# Autodesk Inventor assembly: UBG-Antrieb
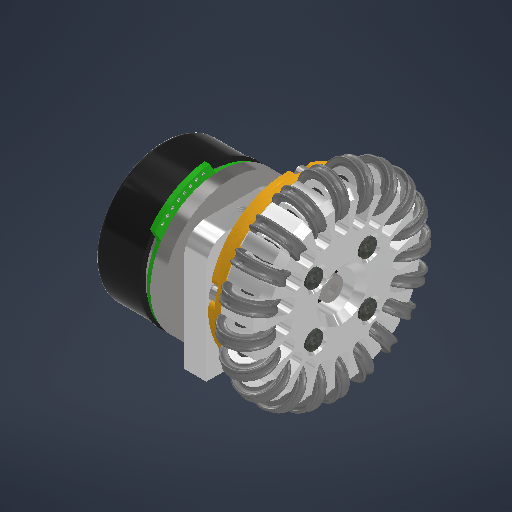
[picture p0: Inventor's stored thumbnail of the model, 512x512]
Saved by Autodesk Inventor 2025.2 (Build 292293000, 293)
## iProperties
Created: 2024-11-07
Part Number: UBG-Antrieb
Document SubType Name: Assembly
Designer: Fabian
Author: Fabian
## Documents named in this file (8)
- C:\Users\Faabs\Desktop\HBG v2025\Oberbaugruppen\OBG-Antrieb\OBG-Antrieb.iam
- C:\Users\Faabs\Desktop\HBG v2025\Oberbaugruppen\OBG-Antrieb\Bauteile\Lagerblock.ipt
- C:\Users\Faabs\Desktop\HBG v2025\Oberbaugruppen\OBG-Antrieb\Bauteile\EC45_50W.ipt
- C:\Users\Faabs\Desktop\HBG v2025\Verbindungselemente\DIN 912\DIN 912 - M3 x 0,5 x 6 x 4,75.ipt
- C:\Users\Faabs\Desktop\HBG v2025\Oberbaugruppen\OBG-Antrieb\Bauteile\18z.ipt
- C:\Users\Faabs\Desktop\HBG v2025\Unterbaugruppen\UBG-Rad\UBG-Rad.iam
- C:\Users\Faabs\Desktop\HBG v2025\Verbindungselemente\DIN 912\DIN 912 - M4 x 0,7 x 16 x 14,25.ipt
- C:\Users\Faabs\Desktop\HBG v2025\Verbindungselemente\DIN 125\DIN 125 - A 3,2.ipt
## Components (9 placed, 7 different names)
1. Lagerblock:1 — Passend:1, Passend:2, Passend:3, Einfügen:1, Einfügen:2, Einfügen:3, Passend:5, Fluchtend:2, Einfügen:4
2. EC45_50W:1 — Passend:1, Passend:2, Passend:3, Passend:4, Fluchtend:1
3. 18z:1 — Passend:4, Fluchtend:1
4. UBG-Rad:1 [sub-assembly] — Passend:5, Fluchtend:2
5. DIN 912 - ersetzt durch DIN EN ISO 4762 M3 x 6:1 — Einfügen:1
6. DIN 912 - ersetzt durch DIN EN ISO 4762 M3 x 6:2 — Einfügen:2
7. DIN 912 - ersetzt durch DIN EN ISO 4762 M3 x 6:3 — Einfügen:3
8. DIN 125-1 A A 3,2:1 — Einfügen:4, Einfügen:5
9. DIN 912 - ersetzt durch DIN EN ISO 4762 M4 x 16:1 — Einfügen:5
## Relationships (12: Mate 5, Insert 5, Flush 2)
- Passend:1 [Mate]: Lagerblock:1 ↔ EC45_50W:1
- Passend:2 [Mate]: Lagerblock:1 ↔ EC45_50W:1
- Passend:3 [Mate]: Lagerblock:1 ↔ EC45_50W:1
- Einfügen:1 [Insert]: Lagerblock:1 ↔ DIN 912 - ersetzt durch DIN EN ISO 4762 M3 x 6:1
- Einfügen:2 [Insert]: Lagerblock:1 ↔ DIN 912 - ersetzt durch DIN EN ISO 4762 M3 x 6:2
- Einfügen:3 [Insert]: Lagerblock:1 ↔ DIN 912 - ersetzt durch DIN EN ISO 4762 M3 x 6:3
- Passend:4 [Mate]: EC45_50W:1 ↔ 18z:1
- Fluchtend:1 [Flush] (-0.4 mm): EC45_50W:1 ↔ 18z:1
- Passend:5 [Mate]: Lagerblock:1 ↔ UBG-Rad:1
- Fluchtend:2 [Flush]: Lagerblock:1 ↔ UBG-Rad:1
- Einfügen:4 [Insert]: Lagerblock:1 ↔ DIN 125-1 A A 3,2:1
- Einfügen:5 [Insert]: DIN 125-1 A A 3,2:1 ↔ DIN 912 - ersetzt durch DIN EN ISO 4762 M4 x 16:1
